# Autodesk Inventor assembly: ks
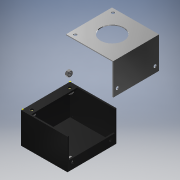
[picture p0: Inventor's stored thumbnail of the model, 180x180]
Saved by Autodesk Inventor 2019 (Build 230136000, 136)
## iProperties
Created: 2020-06-04
Part Number: ks
Material: Genérico
Document SubType Name: Assembly
Designer: eliane
Author: eliane
## Documents named in this file (4)
- C:\Users\Carmo\Desktop\baja\ks.iam
- C:\Users\Carmo\Desktop\joão fazendo a gente de corno\fixaçãoChaveGeral1.ipt
- C:\Users\Carmo\Desktop\joão fazendo a gente de corno\ks2.ipt
- C:\Users\Carmo\Documents\Inventor\Content Center Files\R2019\pt-BR\AS 1112 (2)\AS 1112 - M6  Tipo 10.ipt
## Components (6 placed, 3 different names)
1. fixaçãoChaveGeral1:1 — Alinhamento:1
2. ks2:1 — Alinhamento:1, Coincidência:1, Coincidência:2, Coincidência:3, Coincidência:4, Coincidência:5, Coincidência:6
3. AS 1112 (2) - Métrica M6  Tipo 10:1
4. AS 1112 (2) - Métrica M6  Tipo 10:2 — Coincidência:5, Coincidência:6
5. AS 1112 (2) - Métrica M6  Tipo 10:3 — Coincidência:1, Coincidência:2
6. AS 1112 (2) - Métrica M6  Tipo 10:4 — Coincidência:3, Coincidência:4
## Relationships (7: Mate 6, Flush 1)
- Alinhamento:1 [Flush]: fixaçãoChaveGeral1:1 ↔ ks2:1
- Coincidência:1 [Mate]: ks2:1 ↔ AS 1112 (2) - Métrica M6  Tipo 10:3
- Coincidência:2 [Mate]: ks2:1 ↔ AS 1112 (2) - Métrica M6  Tipo 10:3
- Coincidência:3 [Mate]: ks2:1 ↔ AS 1112 (2) - Métrica M6  Tipo 10:4
- Coincidência:4 [Mate]: ks2:1 ↔ AS 1112 (2) - Métrica M6  Tipo 10:4
- Coincidência:5 [Mate]: ks2:1 ↔ AS 1112 (2) - Métrica M6  Tipo 10:2
- Coincidência:6 [Mate]: ks2:1 ↔ AS 1112 (2) - Métrica M6  Tipo 10:2
